# Autodesk Inventor assembly: MultiPass0V-OnlyRays-V2
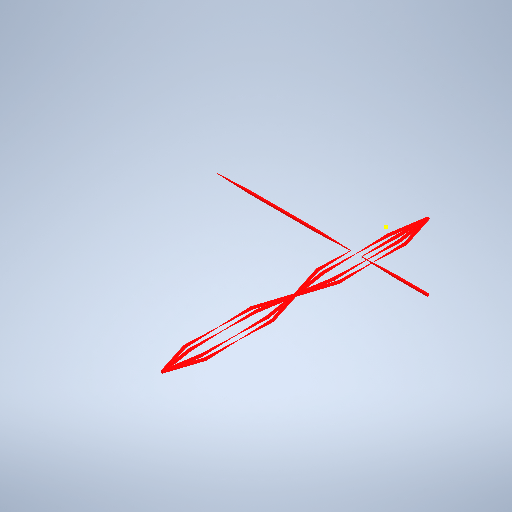
[picture p0: Inventor's stored thumbnail of the model, 512x512]
Saved by Autodesk Inventor 2025 (Build 290162010, 162A)
## iProperties
Created: 2024-08-19
Part Number: MultiPass0V-OnlyRays-V2
Document SubType Name: Assembly
Designer: User
Author: User
## Documents named in this file (9)
- C:\Users\User\Desktop\Hari_Laptop_Contents\KerlinLab\KTN\Multipass\MechanicalDrawing\MultiPass0V-OnlyRays-V2.iam
- C:\Users\User\Desktop\Hari_Laptop_Contents\KerlinLab\KTN\Multipass\MechanicalDrawing\LaserBeamEntry1.ipt
- C:\Users\User\Desktop\Hari_Laptop_Contents\KerlinLab\KTN\Multipass\MechanicalDrawing\EntryMirror.ipt
- C:\Users\User\Desktop\Hari_Laptop_Contents\KerlinLab\KTN\Multipass\MechanicalDrawing\LaserBeamEntry2.ipt
- C:\Users\User\Desktop\Hari_Laptop_Contents\KerlinLab\KTN\Multipass\MechanicalDrawing\LaserBeamCenter1.ipt
- C:\Users\User\Desktop\Hari_Laptop_Contents\KerlinLab\KTN\Multipass\MechanicalDrawing\LaserBeamMirrorAngle1.ipt
- C:\Users\User\Desktop\Hari_Laptop_Contents\KerlinLab\KTN\Multipass\MechanicalDrawing\LaserBeamCenter2.ipt
- C:\Users\User\Desktop\Hari_Laptop_Contents\KerlinLab\KTN\Multipass\MechanicalDrawing\LaserBeamMirrorAngle2.ipt
- C:\Users\User\Desktop\Hari_Laptop_Contents\KerlinLab\KTN\Multipass\MechanicalDrawing\LoopPlane1.ipt
## Components (35 placed, 8 different names)
1. LaserBeamEntry1:1
2. LaserBeamEntry1:2 — Flush:6, Mate:70
3. EntryMirror:1 — Mate:36, Flush:4
4. LaserBeamEntry2:1 — Mate:35
5. LaserBeamEntry2:2 — Mate:37, Flush:6
6. LaserBeamEntry2:3
7. LaserBeamEntry2:4
8. LaserBeamCenter1:1 — Mate:46
9. LaserBeamEntry2:5
10. LaserBeamEntry2:6 — Mate:62
11. LaserBeamEntry2:8
12. LaserBeamEntry2:9
13. LaserBeamEntry2:10
14. LaserBeamCenter1:2 — Mate:58
15. LaserBeamEntry2:11 — Mate:62
16. LaserBeamMirrorAngle1:1 — Mate:67, Mate:101
17. LaserBeamMirrorAngle1:2 — Mate:67
18. LaserBeamMirrorAngle1:3 — Mate:70, Mate:118
19. LaserBeamEntry2:12
20. LaserBeamEntry2:13
21. LaserBeamEntry2:14
22. LaserBeamEntry2:15
23. LaserBeamEntry2:16 — Mate:120
24. LaserBeamEntry2:17
25. LaserBeamEntry2:18 — Mate:93
26. LaserBeamCenter2:1 — Mate:91
27. LaserBeamCenter2:2 — Mate:90, Mate:93
28. LaserBeamEntry2:19 — Mate:119, Mate:120
29. LaserBeamMirrorAngle2:1 — Mate:101, Mate:103
30. LaserBeamMirrorAngle2:2 — Mate:103
31. LaserBeamCenter1:3 — Mate:111
32. LaserBeamEntry2:20 — Mate:111
33. LoopPlane1:1 — Mate:113
34. LaserBeamMirrorAngle2:3
35. LaserBeamMirrorAngle1:4 — Mate:118
## Relationships (24: Mate 22, Flush 2)
- Mate:22
- Mate:23
- Mate:24
- Mate:25
- Mate:35: LaserBeamEntry2:1
- Mate:36: EntryMirror:1
- Flush:4: EntryMirror:1
- Mate:37: LaserBeamEntry2:2
- Flush:6: LaserBeamEntry1:2 ↔ LaserBeamEntry2:2
- Mate:46: LaserBeamCenter1:1
- Mate:58: LaserBeamCenter1:2
- Mate:62: LaserBeamEntry2:6 ↔ LaserBeamEntry2:11
- Mate:67: LaserBeamMirrorAngle1:1 ↔ LaserBeamMirrorAngle1:2
- Mate:70: LaserBeamEntry1:2 ↔ LaserBeamMirrorAngle1:3
- Mate:90: LaserBeamCenter2:2
- Mate:91: LaserBeamCenter2:1
- Mate:93 (0.5 mm): LaserBeamEntry2:18 ↔ LaserBeamCenter2:2
- Mate:101: LaserBeamMirrorAngle1:1 ↔ LaserBeamMirrorAngle2:1
- Mate:103: LaserBeamMirrorAngle2:1 ↔ LaserBeamMirrorAngle2:2
- Mate:111: LaserBeamCenter1:3 ↔ LaserBeamEntry2:20
- Mate:113: LoopPlane1:1
- Mate:118: LaserBeamMirrorAngle1:3 ↔ LaserBeamMirrorAngle1:4
- Mate:119: LaserBeamEntry2:19
- Mate:120: LaserBeamEntry2:16 ↔ LaserBeamEntry2:19
